# Autodesk Inventor assembly: DriveTrain_FrameAssembly
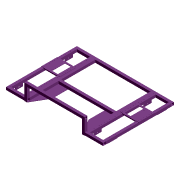
[picture p0: Inventor's stored thumbnail of the model, 180x180]
Saved by Autodesk Inventor 2012 (Build 160160000, 160)
## iProperties
Created: 2012-01-07
Part Number: DriveTrain_FrameAssembly
Document SubType Name: Assembly
Designer: JesseK
Mass: 4481.62 g
Surface Area: 13912.3 cm^2
Volume: 1653.73 cm^3
Density: 2.71 g/cm^3
Author: JesseK
## Documents named in this file (11)
- Z:\UserData\Documents\Inventor\team1885frc\Robot2012\DriveTrain\DriveTrain_FrameAssembly.iam
- Z:\UserData\Documents\Inventor\team1885frc\Robot2012\DriveTrain\DriveTrain_SideRail.ipt
- Z:\UserData\Documents\Inventor\team1885frc\Robot2012\DriveTrain\RearFrameRail.ipt
- Z:\UserData\Documents\Inventor\team1885frc\Robot2012\DriveTrain\FrontBumperRail.ipt
- Z:\UserData\Documents\Inventor\team1885frc\Robot2012\DriveTrain\Frame_SideRail_Inner_2x1.ipt
- Z:\UserData\Documents\Inventor\team1885frc\Robot2012\DriveTrain\WheelBlockMount.ipt
- Z:\UserData\Documents\Inventor\team1885frc\Robot2012\DriveTrain\DriveTrain_MotorMount.ipt
- Z:\UserData\Documents\Inventor\team1885frc\Robot2012\DriveTrain\Frame_FrontCrossRail.ipt
- Z:\UserData\Documents\Inventor\team1885frc\Robot2012\DriveTrain\Frame_FrontVerticalSupport_forFrontCrossbar.ipt
- Z:\UserData\Documents\Inventor\team1885frc\Robot2012\DriveTrain\Frame_MidCrossRail.ipt
- Z:\UserData\Documents\Inventor\team1885frc\Robot2012\Conveyor\Conveyor_Frame_BottomStabilizerPlate.ipt
## Components (23 placed, 10 different names)
1. DriveTrain_SideRail:1 — Flush:1, Flush:2, Mate:1, Flush:4, Mate:2, Flush:5, Flush:6, Mate:3, Mate:11, Mate:18, Mate:19, Mate:20, Mate:23, Mate:24
2. Frame_SideRail_Inner_2x1:1 — Flush:1, Flush:2, Mate:1, Flush:3, Mate:12, Mate:17, Mate:21, Mate:22, Mate:25, Mate:26, Mate:37, Mate:50, Flush:14, Flush:17, Mate:56, Mate:63, Mate:64
3. FrontBumperRail:1 — Flush:3, Flush:4, Mate:2, Mate:51, Flush:18, Mate:57
4. RearFrameRail:1 — Flush:5, Flush:6, Mate:3, Mate:4, Flush:7, Flush:11, Mate:8, Mate:9
5. Frame_SideRail_Inner_2x1:2 — Mate:4, Flush:7, Flush:9, Flush:10, Mate:7, Mate:10, Mate:13, Mate:15, Mate:27, Mate:28, Mate:31, Mate:32, Mate:35, Mate:48, Flush:13, Mate:54, Mate:58, Mate:60, Mate:61
6. FrontBumperRail:2 — Flush:9, Flush:10, Mate:7, Mate:10, Mate:52, Mate:55, Flush:19, Mate:59
7. DriveTrain_SideRail:2 — Flush:11, Mate:8, Mate:9, Mate:14, Mate:16, Mate:29, Mate:30, Mate:33, Mate:34, Mate:62
8. WheelBlockMount:1 — Mate:16, Mate:33, Mate:34
9. WheelBlockMount:2 — Mate:17, Mate:21, Mate:22
10. WheelBlockMount:3 — Mate:18, Mate:19, Mate:20
11. WheelBlockMount:4 — Mate:13, Mate:27, Mate:28
12. WheelBlockMount:5 — Mate:11, Mate:23, Mate:24
13. WheelBlockMount:6 — Mate:12, Mate:25, Mate:26
14. WheelBlockMount:7 — Mate:15, Mate:31, Mate:32
15. WheelBlockMount:8 — Mate:14, Mate:29, Mate:30
16. DriveTrain_MotorMount:1 — Mate:35, Mate:60, Mate:61, Mate:62
17. DriveTrain_MotorMount:2 — Mate:37, Mate:63, Mate:64
18. Frame_FrontVerticalSupport_forFrontCrossbar:1 — Mate:48, Flush:13, Mate:52
19. Frame_FrontVerticalSupport_forFrontCrossbar:2 — Mate:50, Flush:14, Mate:51, Flush:15, Flush:16, Mate:53
20. Frame_FrontCrossRail:2 — Flush:15, Flush:16, Mate:53
21. Frame_MidCrossRail:1 — Flush:17, Mate:54, Mate:55
22. Conveyor_Frame_BottomStabilizerPlate:1 — Mate:56, Flush:18, Mate:57
23. Conveyor_Frame_BottomStabilizerPlate:2 — Mate:58, Flush:19, Mate:59
## Relationships (67: Mate 50, Flush 17)
- Flush:1: DriveTrain_SideRail:1 ↔ Frame_SideRail_Inner_2x1:1
- Flush:2: DriveTrain_SideRail:1 ↔ Frame_SideRail_Inner_2x1:1
- Mate:1 (127 mm): DriveTrain_SideRail:1 ↔ Frame_SideRail_Inner_2x1:1
- Flush:3: Frame_SideRail_Inner_2x1:1 ↔ FrontBumperRail:1
- Flush:4: DriveTrain_SideRail:1 ↔ FrontBumperRail:1
- Mate:2: DriveTrain_SideRail:1 ↔ FrontBumperRail:1
- Flush:5: DriveTrain_SideRail:1 ↔ RearFrameRail:1
- Flush:6: DriveTrain_SideRail:1 ↔ RearFrameRail:1
- Mate:3: DriveTrain_SideRail:1 ↔ RearFrameRail:1
- Mate:4: RearFrameRail:1 ↔ Frame_SideRail_Inner_2x1:2
- Flush:7: RearFrameRail:1 ↔ Frame_SideRail_Inner_2x1:2
- Flush:9: Frame_SideRail_Inner_2x1:2 ↔ FrontBumperRail:2
- Flush:10: Frame_SideRail_Inner_2x1:2 ↔ FrontBumperRail:2
- Mate:7: Frame_SideRail_Inner_2x1:2 ↔ FrontBumperRail:2
- Flush:11: RearFrameRail:1 ↔ DriveTrain_SideRail:2
- Mate:8: RearFrameRail:1 ↔ DriveTrain_SideRail:2
- Mate:9: RearFrameRail:1 ↔ DriveTrain_SideRail:2
- Mate:10: Frame_SideRail_Inner_2x1:2 ↔ FrontBumperRail:2
- Mate:11: DriveTrain_SideRail:1 ↔ WheelBlockMount:5
- Mate:12: Frame_SideRail_Inner_2x1:1 ↔ WheelBlockMount:6
- Mate:13: Frame_SideRail_Inner_2x1:2 ↔ WheelBlockMount:4
- Mate:14: DriveTrain_SideRail:2 ↔ WheelBlockMount:8
- Mate:15: Frame_SideRail_Inner_2x1:2 ↔ WheelBlockMount:7
- Mate:16: DriveTrain_SideRail:2 ↔ WheelBlockMount:1
- Mate:17: Frame_SideRail_Inner_2x1:1 ↔ WheelBlockMount:2
- Mate:18: DriveTrain_SideRail:1 ↔ WheelBlockMount:3
- Mate:19: DriveTrain_SideRail:1 ↔ WheelBlockMount:3
- Mate:20: DriveTrain_SideRail:1 ↔ WheelBlockMount:3
- Mate:21: Frame_SideRail_Inner_2x1:1 ↔ WheelBlockMount:2
- Mate:22: Frame_SideRail_Inner_2x1:1 ↔ WheelBlockMount:2
- Mate:23: DriveTrain_SideRail:1 ↔ WheelBlockMount:5
- Mate:24: DriveTrain_SideRail:1 ↔ WheelBlockMount:5
- Mate:25: Frame_SideRail_Inner_2x1:1 ↔ WheelBlockMount:6
- Mate:26: Frame_SideRail_Inner_2x1:1 ↔ WheelBlockMount:6
- Mate:27: Frame_SideRail_Inner_2x1:2 ↔ WheelBlockMount:4
- Mate:28: Frame_SideRail_Inner_2x1:2 ↔ WheelBlockMount:4
- Mate:29: DriveTrain_SideRail:2 ↔ WheelBlockMount:8
- Mate:30: DriveTrain_SideRail:2 ↔ WheelBlockMount:8
- Mate:31: Frame_SideRail_Inner_2x1:2 ↔ WheelBlockMount:7
- Mate:32: Frame_SideRail_Inner_2x1:2 ↔ WheelBlockMount:7
- Mate:33: DriveTrain_SideRail:2 ↔ WheelBlockMount:1
- Mate:34: DriveTrain_SideRail:2 ↔ WheelBlockMount:1
- Mate:35: Frame_SideRail_Inner_2x1:2 ↔ DriveTrain_MotorMount:1
- Mate:37: Frame_SideRail_Inner_2x1:1 ↔ DriveTrain_MotorMount:2
- Mate:48: Frame_SideRail_Inner_2x1:2 ↔ Frame_FrontVerticalSupport_forFrontCrossbar:1
- Flush:13: Frame_SideRail_Inner_2x1:2 ↔ Frame_FrontVerticalSupport_forFrontCrossbar:1
- Mate:50: Frame_SideRail_Inner_2x1:1 ↔ Frame_FrontVerticalSupport_forFrontCrossbar:2
- Flush:14: Frame_SideRail_Inner_2x1:1 ↔ Frame_FrontVerticalSupport_forFrontCrossbar:2
- Mate:51: FrontBumperRail:1 ↔ Frame_FrontVerticalSupport_forFrontCrossbar:2
- Mate:52: FrontBumperRail:2 ↔ Frame_FrontVerticalSupport_forFrontCrossbar:1
- Flush:15: Frame_FrontVerticalSupport_forFrontCrossbar:2 ↔ Frame_FrontCrossRail:2
- Flush:16: Frame_FrontVerticalSupport_forFrontCrossbar:2 ↔ Frame_FrontCrossRail:2
- Mate:53: Frame_FrontVerticalSupport_forFrontCrossbar:2 ↔ Frame_FrontCrossRail:2
- Flush:17: Frame_SideRail_Inner_2x1:1 ↔ Frame_MidCrossRail:1
- Mate:54: Frame_SideRail_Inner_2x1:2 ↔ Frame_MidCrossRail:1
- Mate:55 (304.8 mm): FrontBumperRail:2 ↔ Frame_MidCrossRail:1
- Mate:56: Frame_SideRail_Inner_2x1:1 ↔ Conveyor_Frame_BottomStabilizerPlate:1
- Flush:18: FrontBumperRail:1 ↔ Conveyor_Frame_BottomStabilizerPlate:1
- Mate:57: FrontBumperRail:1 ↔ Conveyor_Frame_BottomStabilizerPlate:1
- Mate:58: Frame_SideRail_Inner_2x1:2 ↔ Conveyor_Frame_BottomStabilizerPlate:2
- Flush:19: FrontBumperRail:2 ↔ Conveyor_Frame_BottomStabilizerPlate:2
- Mate:59: FrontBumperRail:2 ↔ Conveyor_Frame_BottomStabilizerPlate:2
- Mate:60: Frame_SideRail_Inner_2x1:2 ↔ DriveTrain_MotorMount:1
- Mate:61: Frame_SideRail_Inner_2x1:2 ↔ DriveTrain_MotorMount:1
- Mate:62: DriveTrain_SideRail:2 ↔ DriveTrain_MotorMount:1
- Mate:63: Frame_SideRail_Inner_2x1:1 ↔ DriveTrain_MotorMount:2
- Mate:64: Frame_SideRail_Inner_2x1:1 ↔ DriveTrain_MotorMount:2
